# Autodesk Inventor assembly: battery
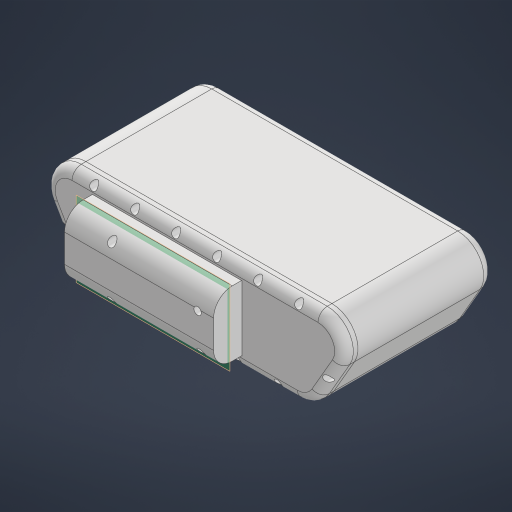
[picture p0: Inventor's stored thumbnail of the model, 512x512]
Saved by Autodesk Inventor 2024 (Build 280153000, 153)
## iProperties
Created: 2024-05-04
Part Number: battery
Document SubType Name: Assembly
Designer: markm
Author: markm
## Documents named in this file (5)
- C:\Users\markm\OneDrive\Документы\Inventor\eventide\back\battery\battery.iam
- C:\Users\markm\OneDrive\Документы\Inventor\eventide\back\battery\cell.ipt
- C:\Users\markm\OneDrive\Документы\Inventor\eventide\back\battery\frame.ipt
- C:\Users\markm\OneDrive\Документы\Inventor\eventide\back\battery\box.ipt
- C:\Users\markm\OneDrive\Документы\Inventor\eventide\back\battery\Part3.ipt
## Components (16 placed, 4 different names)
1. frame:1 — Mate:1, Mate:2, Flush:4, Flush:5, Mate:3, Mate:4, Mate:5
2. cell:2 — Mate:2, Flush:5
3. box:1 — Mate:3, Mate:4, Mate:5
4. Part3:1
5. cell:1 — Mate:1, Flush:4
6. cell:3
7. cell:4
8. cell:5
9. cell:6
10. cell:7
11. cell:8
12. cell:9
13. cell:10
14. cell:11
15. cell:12
16. cell:13
## Component patterns: (12 elements, first: cell:1)
## Relationships (7: Mate 5, Flush 2)
- Mate:1: frame:1 ↔ cell:1
- Mate:2: frame:1 ↔ cell:2
- Flush:4: frame:1 ↔ cell:1
- Flush:5: frame:1 ↔ cell:2
- Mate:3: frame:1 ↔ box:1
- Mate:4: frame:1 ↔ box:1
- Mate:5 (0.25 mm): frame:1 ↔ box:1
